# Autodesk Inventor assembly: Partical Launcher
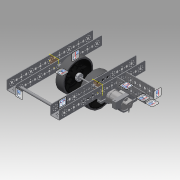
[picture p0: Inventor's stored thumbnail of the model, 180x180]
Saved by Autodesk Inventor 2016 (Build 200138000, 138)
## iProperties
Created: 2016-09-20
Part Number: Partical Launcher
Document SubType Name: Assembly
Designer: Delta
Author: Delta
## Documents named in this file (10)
- C:\Robotics\2016-17_CAD\Partical Launcher.iam
- C:\Robotics\CAD\2015-16\COTSParts\Tetrix\Tetrix channel 288mm.ipt
- C:\Robotics\CAD\2015-16\custom cad parts\particle_launcher_Tube.ipt
- C:\Robotics\CAD\2015-16\COTSParts\Tetrix\Tetrix channel 96mm.ipt
- C:\Robotics\CAD\2015-16\COTSParts\Tetrix\Tetrix motor_MIR1.ipt
- C:\Robotics\CAD\2015-16\COTSParts\Tetrix\Tetrix motor mount_MIR1.ipt
- C:\Robotics\CAD\2015-16\COTSParts\Wheels\Andymark Stealth Wheelam-2648_4inWheel8mmHub (1).iam
- C:\Robotics\CAD\2015-16\COTSParts\Tetrix\Tetrix hub - motor.ipt
- C:\Robotics\CAD\2015-16\COTSParts\Tetrix\Tetrix shaft 250mm.ipt
- C:\Robotics\CAD\2015-16\COTSParts\Tetrix\Tetrix shaft collar.ipt
## Components (17 placed, 9 different names)
1. Tetrix motor mount_MIR1:1 — Insert:4, Insert:5
2. Tetrix channel 288mm:1 — Flush:1, Flush:2, Mate:1, Insert:2, Flush:3, Flush:4, Flush:5, Insert:5, Insert:9, Insert:10
3. Tetrix channel 288mm:2 — Flush:1, Flush:2, Mate:1, Insert:1, Insert:8, Insert:11, Insert:12
4. particle_launcher_Tube:1 — Insert:1, Insert:2
5. Tetrix channel 96mm:1 — Flush:3, Flush:4, Flush:5
6. Tetrix motor_MIR1:2
7. Tetrix motor_MIR1:3 — Insert:3, Insert:4, Insert:6
8. Tetrix motor mount_MIR1:2 — Insert:3
9. Andymark Stealth Wheelam-2648_4inWheel8mmHub (1):1 [sub-assembly] — Insert:7
10. Andymark Stealth Wheelam-2648_4inWheel8mmHub (1):2 [sub-assembly] — Insert:13
11. Tetrix hub - motor:1 — Insert:6, Insert:7
12. Tetrix hub - motor:2 — Insert:13, Insert:14
13. Tetrix shaft 250mm:2 — Insert:8, Insert:14
14. Tetrix shaft collar:1 — Insert:11
15. Tetrix shaft collar:2 — Insert:12
16. Tetrix shaft collar:3 — Insert:10
17. Tetrix shaft collar:4 — Insert:9
## Relationships (20: Insert 14, Flush 5, Mate 1)
- Flush:1: Tetrix channel 288mm:1 ↔ Tetrix channel 288mm:2
- Flush:2: Tetrix channel 288mm:1 ↔ Tetrix channel 288mm:2
- Mate:1 (114.3 mm): Tetrix channel 288mm:1 ↔ Tetrix channel 288mm:2
- Insert:1: Tetrix channel 288mm:2 ↔ particle_launcher_Tube:1
- Insert:2: Tetrix channel 288mm:1 ↔ particle_launcher_Tube:1
- Flush:3 (-95.504 mm): Tetrix channel 288mm:1 ↔ Tetrix channel 96mm:1
- Flush:4: Tetrix channel 288mm:1 ↔ Tetrix channel 96mm:1
- Flush:5: Tetrix channel 288mm:1 ↔ Tetrix channel 96mm:1
- Insert:3: Tetrix motor_MIR1:3 ↔ Tetrix motor mount_MIR1:2
- Insert:4 (-12.7 mm): Tetrix motor mount_MIR1:1 ↔ Tetrix motor_MIR1:3
- Insert:5: Tetrix motor mount_MIR1:1 ↔ Tetrix channel 288mm:1
- Insert:6: Tetrix motor_MIR1:3 ↔ Tetrix hub - motor:1
- Insert:7: Andymark Stealth Wheelam-2648_4inWheel8mmHub (1):1 ↔ Tetrix hub - motor:1
- Insert:8 (-15.24 mm): Tetrix channel 288mm:2 ↔ Tetrix shaft 250mm:2
- Insert:9: Tetrix channel 288mm:1 ↔ Tetrix shaft collar:4
- Insert:10: Tetrix channel 288mm:1 ↔ Tetrix shaft collar:3
- Insert:11: Tetrix channel 288mm:2 ↔ Tetrix shaft collar:1
- Insert:12: Tetrix channel 288mm:2 ↔ Tetrix shaft collar:2
- Insert:13: Andymark Stealth Wheelam-2648_4inWheel8mmHub (1):2 ↔ Tetrix hub - motor:2
- Insert:14 (-86.36 mm): Tetrix hub - motor:2 ↔ Tetrix shaft 250mm:2
